# Autodesk Inventor assembly: motor assembly
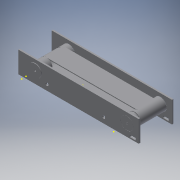
[picture p0: Inventor's stored thumbnail of the model, 180x180]
Saved by Autodesk Inventor 2019 (Build 230136000, 136)
## iProperties
Created: 2020-03-01
Part Number: motor assembly
Document SubType Name: Assembly
Designer: Hp
Author: Hp
## Documents named in this file (5)
- C:\Users\Hp\Documents\autodesk\explo\motor assembly.iam
- C:\Users\Hp\Documents\autodesk\explo\a\motor holde 2.ipt
- C:\Users\Hp\Documents\autodesk\explo\a\motor holder.ipt
- C:\Users\Hp\Documents\autodesk\explo\s\conveyor belt.ipt
- C:\Users\Hp\Documents\autodesk\explo\s\dc motor.ipt
## Components (9 placed, 4 different names)
1. motor holde 2:1 — Rotational:2, Rotational:3
2. motor holde 2:2 — Rotational:4, Rotational:5
3. motor holde 2:3 — Rotational:5
4. motor holder:1 — Rotational:8
5. motor holder:2 — Rotational:3, Rotational:4
6. conveyor belt:1 — Rotational:1, Rotational:6, Rotational:7
7. dc motor:1 — Rotational:1, Rotational:2
8. motor holde 2:4 — Rotational:7, Rotational:8
9. motor holde 2:5 — Rotational:6
## Relationships (8: RevoluteJoint 8)
- Rotational:1 [RevoluteJoint] (-30.1625 mm): conveyor belt:1 ↔ dc motor:1
- Rotational:2 [RevoluteJoint]: motor holde 2:1 ↔ dc motor:1
- Rotational:3 [RevoluteJoint]: motor holde 2:1 ↔ motor holder:2
- Rotational:4 [RevoluteJoint] (-1.5875 mm): motor holde 2:2 ↔ motor holder:2
- Rotational:5 [RevoluteJoint] (14.2875 mm): motor holde 2:2 ↔ motor holde 2:3
- Rotational:6 [RevoluteJoint] (-14.2875 mm): conveyor belt:1 ↔ motor holde 2:5
- Rotational:7 [RevoluteJoint] (-14.2875 mm): conveyor belt:1 ↔ motor holde 2:4
- Rotational:8 [RevoluteJoint]: motor holder:1 ↔ motor holde 2:4
